# Autodesk Inventor assembly: Assembly_Omniscope_v1
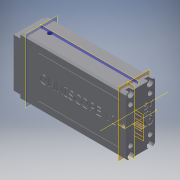
[picture p0: Inventor's stored thumbnail of the model, 180x180]
Saved by Autodesk Inventor 2019.4 (Build 234330000, 330)
## iProperties
Created: 2021-09-22
Part Number: Assembly_Omniscope_v1
Material: Generisch
Document SubType Name: Assembly
Designer: Muriel
Mass: 21.4058 g
Surface Area: 211.771 cm^2
Volume: 21.4058 cm^3
Density: 1 g/cm^3
Author: Muriel
## Documents named in this file (9)
- C:\Users\diederichbenedict\Dropbox\Dokumente\Promotion\PROJECTS\Omniscope\INVENTOR\Assembly_Omniscope_v1.iam
- C:\Users\diederichbenedict\Dropbox\Dokumente\Promotion\PROJECTS\Omniscope\INVENTOR\01_Camera_Module_left_v0.ipt
- C:\Users\diederichbenedict\Dropbox\Dokumente\Promotion\PROJECTS\Omniscope\INVENTOR\01_Camera_Module_Lit.ipt
- C:\Users\diederichbenedict\Dropbox\Dokumente\Promotion\PROJECTS\Omniscope\INVENTOR\00_ESP32_Board.ipt
- C:\Users\diederichbenedict\Dropbox\Dokumente\Promotion\PROJECTS\Omniscope\INVENTOR\03_Camera_Clip.ipt
- C:\Users\diederichbenedict\Dropbox\Dokumente\Promotion\PROJECTS\Omniscope\INVENTOR\02_Camera_Lid.ipt
- C:\Users\diederichbenedict\Dropbox\Dokumente\Promotion\PROJECTS\Omniscope\INVENTOR\00_OV_lens.ipt
- C:\Users\diederichbenedict\Dropbox\Dokumente\Promotion\PROJECTS\Omniscope\INVENTOR\Omnivision_Objectivelens_mount.ipt
- C:\Users\diederichbenedict\Dropbox\Dokumente\Promotion\PROJECTS\Omniscope\INVENTOR\00_Pinhead_2.54_5x_male.ipt
## Components (10 placed, 8 different names)
1. 01_Camera_Module_left_v0:1 — Fluchtend:2, Einfügen:2, Fluchtend:3, Einfügen:3, Fluchtend:4, Fluchtend:5, Insert:5, Flush:6, Flush:7
2. 01_Camera_Module_Lit:1 — Fluchtend:2
3. 00_ESP32_Board:1 — Einfügen:2, Insert:4
4. 00_ESP32_Board:2 — Einfügen:3
5. 03_Camera_Clip:1 — Fluchtend:3
6. 02_Camera_Lid:1 — Fluchtend:4, Fluchtend:5, Flush:8, Flush:9, Flush:10
7. 00_OV_lens:1 — Insert:4
8. 00_OV_lens:2 — Insert:5
9. Omnivision_Objectivelens_mount:1 — Flush:6, Flush:7
10. 00_Pinhead_2.54_5x_male:1 — Flush:8, Flush:9, Flush:10
## Relationships (13: Flush 9, Insert 4)
- Fluchtend:2 [Flush]: 01_Camera_Module_left_v0:1 ↔ 01_Camera_Module_Lit:1
- Einfügen:2 [Insert]: 01_Camera_Module_left_v0:1 ↔ 00_ESP32_Board:1
- Fluchtend:3 [Flush]: 01_Camera_Module_left_v0:1 ↔ 03_Camera_Clip:1
- Einfügen:3 [Insert]: 01_Camera_Module_left_v0:1 ↔ 00_ESP32_Board:2
- Fluchtend:4 [Flush]: 01_Camera_Module_left_v0:1 ↔ 02_Camera_Lid:1
- Fluchtend:5 [Flush]: 01_Camera_Module_left_v0:1 ↔ 02_Camera_Lid:1
- Insert:4 (-8 mm): 00_ESP32_Board:1 ↔ 00_OV_lens:1
- Insert:5 (-8 mm): 01_Camera_Module_left_v0:1 ↔ 00_OV_lens:2
- Flush:6: 01_Camera_Module_left_v0:1 ↔ Omnivision_Objectivelens_mount:1
- Flush:7: 01_Camera_Module_left_v0:1 ↔ Omnivision_Objectivelens_mount:1
- Flush:8: 02_Camera_Lid:1 ↔ 00_Pinhead_2.54_5x_male:1
- Flush:9: 02_Camera_Lid:1 ↔ 00_Pinhead_2.54_5x_male:1
- Flush:10: 02_Camera_Lid:1 ↔ 00_Pinhead_2.54_5x_male:1
